# Autodesk Inventor assembly: prototype
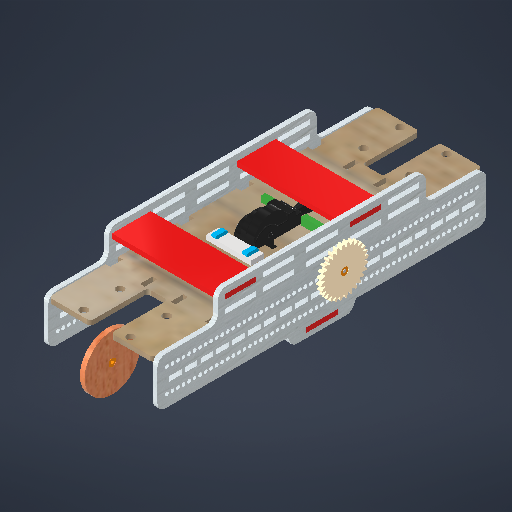
[picture p0: Inventor's stored thumbnail of the model, 512x512]
Saved by Autodesk Inventor 2025.3 (Build 293356030, 356C)
## iProperties
Created: 2025-09-04
Part Number: prototype
Document SubType Name: Assembly
Designer: 陳泓任
Author: 陳泓任
## Documents named in this file (11)
- C:\Users\Ou918\3D-model-temp\introduction to mechanical engineering(1)\version_4\prototype.iam
- C:\Users\Ou918\3D-model-temp\introduction to mechanical engineering(1)\發條組合\發條組合.iam
- C:\Users\Ou918\3D-model-temp\introduction to mechanical engineering(1)\version_2\plug.ipt
- C:\Users\Ou918\3D-model-temp\introduction to mechanical engineering(1)\beam.ipt
- C:\Users\Ou918\3D-model-temp\introduction to mechanical engineering(1)\big gear(with sleeve).iam
- C:\Users\Ou918\3D-model-temp\introduction to mechanical engineering(1)\35mm wheel(with sleeve).iam
- C:\Users\Ou918\3D-model-temp\introduction to mechanical engineering(1)\baffle.ipt
- C:\Users\Ou918\3D-model-temp\introduction to mechanical engineering(1)\support.ipt
- C:\Users\Ou918\3D-model-temp\introduction to mechanical engineering(1)\version_3\support.ipt
- C:\Users\Ou918\3D-model-temp\introduction to mechanical engineering(1)\version_4\side_frame.ipt
- C:\Users\Ou918\3D-model-temp\introduction to mechanical engineering(1)\version_3\main_frame.ipt
## Components (16 placed, 9 different names)
1. main_frame:1 — 貼合:107, 貼合:108, 貼合:109, 貼合:110, 貼合:111, 貼合:112, 貼合:113, 貼合:114, 貼合:115
2. 發條組合:1 [sub-assembly] — gear, 貼合:82, 貼合:90, 貼合:93, 貼合:94, 貼合:114, 貼合:116
3. side_frame:1 — 齊平:6, 貼合:96, 貼合:97
4. side_frame:2 — 貼合:98, 齊平:7, 貼合:99, 齊平:8, 貼合:100, 貼合:101, 貼合:102, 齊平:9, 貼合:103, 角度:2, 貼合:116
5. beam:1 — 齊平:8, 貼合:100, 貼合:101
6. beam:2 — 貼合:102, 齊平:9, 貼合:103
7. beam:3 — 齊平:6, 貼合:96, 貼合:97, 貼合:98, 齊平:7, 貼合:99
8. big gear(with sleeve):1 [sub-assembly] — gear
9. 35mm wheel(with sleeve):3 [sub-assembly]
10. support:3 — 貼合:54, 貼合:75, 貼合:107
11. support:4 — 貼合:53, 貼合:55, 貼合:56, 貼合:57, 貼合:58, 貼合:108, 貼合:109
12. baffle:1 — 貼合:53, 貼合:54, 貼合:55, 貼合:56, 貼合:94, 貼合:110
13. baffle:2 — 貼合:57, 貼合:58, 貼合:75
14. baffle:3 — 貼合:86, 貼合:88, 貼合:89, 貼合:90, 貼合:93
15. plug:3 — 貼合:86, 貼合:113, 貼合:115
16. plug:4 — 貼合:88, 貼合:89, 貼合:112
## Relationships (38: Mate 32, Flush 4, Insert 1, Angle 1)
- gear [Insert]: 發條組合:1 ↔ big gear(with sleeve):1
- 貼合:53 [Mate]: support:4 ↔ baffle:1
- 貼合:54 [Mate]: support:3 ↔ baffle:1
- 貼合:55 [Mate]: support:4 ↔ baffle:1
- 貼合:56 [Mate]: support:4 ↔ baffle:1
- 貼合:57 [Mate]: support:4 ↔ baffle:2
- 貼合:58 [Mate]: support:4 ↔ baffle:2
- 貼合:75 [Mate]: support:3 ↔ baffle:2
- 貼合:82 [Mate] (-6.75 mm): 發條組合:1
- 貼合:86 [Mate]: baffle:3 ↔ plug:3
- 貼合:88 [Mate]: baffle:3 ↔ plug:4
- 貼合:89 [Mate]: baffle:3 ↔ plug:4
- 貼合:90 [Mate]: 發條組合:1 ↔ baffle:3
- 貼合:93 [Mate]: 發條組合:1 ↔ baffle:3
- 貼合:94 [Mate]: 發條組合:1 ↔ baffle:1
- 齊平:6 [Flush]: side_frame:1 ↔ beam:3
- 貼合:96 [Mate]: side_frame:1 ↔ beam:3
- 貼合:97 [Mate]: side_frame:1 ↔ beam:3
- 貼合:98 [Mate]: side_frame:2 ↔ beam:3
- 齊平:7 [Flush]: side_frame:2 ↔ beam:3
- 貼合:99 [Mate]: side_frame:2 ↔ beam:3
- 齊平:8 [Flush]: side_frame:2 ↔ beam:1
- 貼合:100 [Mate]: side_frame:2 ↔ beam:1
- 貼合:101 [Mate]: side_frame:2 ↔ beam:1
- 貼合:102 [Mate]: side_frame:2 ↔ beam:2
- 齊平:9 [Flush]: side_frame:2 ↔ beam:2
- 貼合:103 [Mate]: side_frame:2 ↔ beam:2
- 角度:2 [Angle] (90 deg): side_frame:2
- 貼合:107 [Mate]: main_frame:1 ↔ support:3
- 貼合:108 [Mate]: main_frame:1 ↔ support:4
- 貼合:109 [Mate]: main_frame:1 ↔ support:4
- 貼合:110 [Mate]: main_frame:1 ↔ baffle:1
- 貼合:111 [Mate]: main_frame:1
- 貼合:112 [Mate]: main_frame:1 ↔ plug:4
- 貼合:113 [Mate]: main_frame:1 ↔ plug:3
- 貼合:114 [Mate]: main_frame:1 ↔ 發條組合:1
- 貼合:115 [Mate]: main_frame:1 ↔ plug:3
- 貼合:116 [Mate]: 發條組合:1 ↔ side_frame:2
